# Autodesk Inventor assembly: Chasis
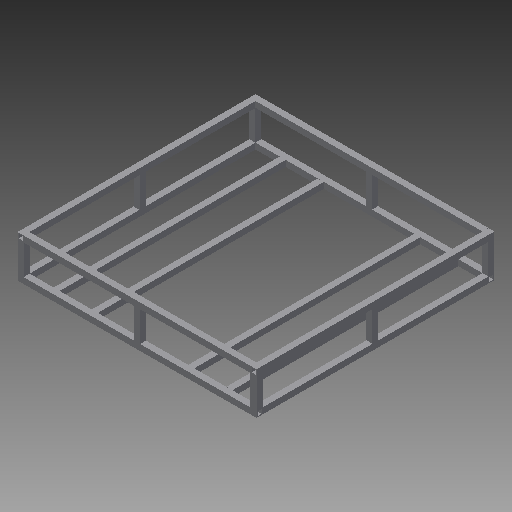
[picture p0: Inventor's stored thumbnail of the model, 512x512]
Saved by Autodesk Inventor 2019 (Build 230136000, 136)
## iProperties
has-driver: False
num-sensors: 0
robot-weight-kg: 226.0
robot-prefer-metric: False
robot-driveTrainType: 3
has-driver: True
driver-type: 1
motor-type: 0
driver-port1: 1
driver-port2: -1
driver-isCan: False
driver-lowerLimit: 0.0
driver-upperLimit: 0.0
driver-inputGear: 0.0
driver-outputGear: 0.0
driver-hasBrake: False
has-wheel: True
wheel-type: 3
wheel-isDriveWheel: True
wheel-frictionLevel: 1
has-pneumatic: False
has-elevator: False
driver-port1: 0
Created: 2019-01-05
Part Number: Chasis
Document SubType Name: Assembly
Designer: Jacob's Laptop
Mass: 1920.36 g
Surface Area: 12177.4 cm^2
Volume: 1920.36 cm^3
Density: 1 g/cm^3
Author: Jacob's Laptop
## Documents named in this file (4)
- D:\Synthesis Robots\Epsilon\Chasis.iam
- D:\Synthesis Robots\Epsilon\Chasis\Chasis Long Length.ipt
- D:\Synthesis Robots\Epsilon\Chasis\Chasis Short Length.ipt
- D:\Synthesis Robots\Epsilon\Chasis\Chasis Hieght.ipt
## Components (20 placed, 3 different names)
1. Chasis Long Length:1 — Mate:1, Flush:1, Flush:2, Mate:2, Flush:3, Flush:4, Mate:3, Flush:5, Flush:6, Mate:6, Flush:12
2. Chasis Long Length:2 — Mate:4, Flush:7, Flush:8, Mate:5, Flush:9, Mate:7, Flush:13, Flush:14
3. Chasis Short Length:1 — Mate:2, Flush:3, Flush:4
4. Chasis Short Length:2 — Mate:3, Flush:5, Flush:6, Mate:4, Flush:7, Flush:8, Flush:10, Flush:11, Flush:24
5. Chasis Hieght:1 — Mate:1, Flush:1, Flush:2, Mate:11, Flush:21, Flush:22, Mate:13, Mate:17
6. Chasis Hieght:2 — Mate:6, Flush:11, Flush:12
7. Chasis Hieght:3 — Mate:5, Flush:9, Flush:10, Mate:15
8. Chasis Hieght:4 — Mate:7, Flush:13, Flush:14, Mate:19
9. Chasis Long Length:3 — Mate:11, Flush:21, Flush:22, Mate:16, Flush:25
10. Chasis Long Length:4 — Mate:14, Mate:21, Flush:27, Mate:22, Flush:28, Mate:23, Flush:29, Mate:24, Flush:30
11. Chasis Short Length:3 — Mate:18, Flush:26, Mate:27
12. Chasis Short Length:4 — Mate:12, Flush:23, Mate:28
13. Chasis Hieght:5 — Mate:18, Flush:26, Mate:19
14. Chasis Hieght:6 — Mate:16, Flush:25, Mate:17
15. Chasis Hieght:7 — Mate:12, Flush:23, Mate:13
16. Chasis Hieght:8 — Mate:14, Flush:24, Mate:15
17. Chasis Short Length:5 — Mate:21, Flush:27, Mate:25, Mate:27
18. Chasis Short Length:6 — Mate:22, Flush:28, Mate:25
19. Chasis Short Length:7 — Mate:23, Flush:29, Mate:26
20. Chasis Short Length:8 — Mate:24, Flush:30, Mate:26, Mate:28
## Relationships (57: Flush 30, Mate 27)
- Mate:1: Chasis Long Length:1 ↔ Chasis Hieght:1
- Flush:1: Chasis Long Length:1 ↔ Chasis Hieght:1
- Flush:2: Chasis Long Length:1 ↔ Chasis Hieght:1
- Mate:2: Chasis Long Length:1 ↔ Chasis Short Length:1
- Flush:3: Chasis Long Length:1 ↔ Chasis Short Length:1
- Flush:4: Chasis Long Length:1 ↔ Chasis Short Length:1
- Mate:3: Chasis Long Length:1 ↔ Chasis Short Length:2
- Flush:5: Chasis Long Length:1 ↔ Chasis Short Length:2
- Flush:6: Chasis Long Length:1 ↔ Chasis Short Length:2
- Mate:4: Chasis Long Length:2 ↔ Chasis Short Length:2
- Flush:7: Chasis Long Length:2 ↔ Chasis Short Length:2
- Flush:8: Chasis Long Length:2 ↔ Chasis Short Length:2
- Mate:5: Chasis Long Length:2 ↔ Chasis Hieght:3
- Flush:9: Chasis Long Length:2 ↔ Chasis Hieght:3
- Flush:10: Chasis Short Length:2 ↔ Chasis Hieght:3
- Mate:6: Chasis Long Length:1 ↔ Chasis Hieght:2
- Flush:11: Chasis Short Length:2 ↔ Chasis Hieght:2
- Flush:12: Chasis Long Length:1 ↔ Chasis Hieght:2
- Mate:7: Chasis Long Length:2 ↔ Chasis Hieght:4
- Flush:13: Chasis Long Length:2 ↔ Chasis Hieght:4
- Flush:14: Chasis Long Length:2 ↔ Chasis Hieght:4
- [Mate]: Chasis Long Length:3 ↔ Chasis Short Length:3
- [Flush]: Chasis Long Length:3 ↔ Chasis Short Length:3
- [Flush]: Chasis Long Length:3 ↔ Chasis Short Length:3
- [Mate]: Chasis Long Length:3 ↔ Chasis Short Length:4
- [Flush]: Chasis Long Length:3 ↔ Chasis Short Length:4
- [Flush]: Chasis Long Length:3 ↔ Chasis Short Length:4
- [Mate]: Chasis Long Length:4 ↔ Chasis Short Length:4
- [Flush]: Chasis Long Length:4 ↔ Chasis Short Length:4
- [Flush]: Chasis Long Length:4 ↔ Chasis Short Length:4
- Mate:11: Chasis Hieght:1 ↔ Chasis Long Length:3
- Flush:21: Chasis Hieght:1 ↔ Chasis Long Length:3
- Flush:22: Chasis Hieght:1 ↔ Chasis Long Length:3
- Mate:12: Chasis Short Length:4 ↔ Chasis Hieght:7
- Flush:23: Chasis Short Length:4 ↔ Chasis Hieght:7
- Mate:13 (349.25 mm): Chasis Hieght:1 ↔ Chasis Hieght:7
- Mate:14: Chasis Long Length:4 ↔ Chasis Hieght:8
- Flush:24: Chasis Short Length:2 ↔ Chasis Hieght:8
- Mate:15 (349.25 mm): Chasis Hieght:3 ↔ Chasis Hieght:8
- Mate:16: Chasis Long Length:3 ↔ Chasis Hieght:6
- Flush:25: Chasis Long Length:3 ↔ Chasis Hieght:6
- Mate:17 (349.25 mm): Chasis Hieght:1 ↔ Chasis Hieght:6
- Mate:18: Chasis Short Length:3 ↔ Chasis Hieght:5
- Flush:26: Chasis Short Length:3 ↔ Chasis Hieght:5
- Mate:19 (349.25 mm): Chasis Hieght:4 ↔ Chasis Hieght:5
- Mate:21: Chasis Long Length:4 ↔ Chasis Short Length:5
- Flush:27: Chasis Long Length:4 ↔ Chasis Short Length:5
- Mate:22: Chasis Long Length:4 ↔ Chasis Short Length:6
- Flush:28: Chasis Long Length:4 ↔ Chasis Short Length:6
- Mate:23: Chasis Long Length:4 ↔ Chasis Short Length:7
- Flush:29: Chasis Long Length:4 ↔ Chasis Short Length:7
- Mate:24: Chasis Long Length:4 ↔ Chasis Short Length:8
- Flush:30: Chasis Long Length:4 ↔ Chasis Short Length:8
- Mate:25 (101.6 mm): Chasis Short Length:5 ↔ Chasis Short Length:6
- Mate:26 (101.6 mm): Chasis Short Length:7 ↔ Chasis Short Length:8
- Mate:27 (76.2 mm): Chasis Short Length:3 ↔ Chasis Short Length:5
- Mate:28 (76.2 mm): Chasis Short Length:4 ↔ Chasis Short Length:8
## Named parameters: d21_d3 = 0 mm, d22_d4 = 0 mm, d23_d5 = 0 mm, d24_d6 = 0 mm, d25_d7 = 0 mm, d26_d8 = 0 mm, d27_d9 = 0 mm, d28_d10 = 0 mm, d29_d11 = 0 mm
